# Autodesk Inventor assembly: 6 Plaction with bearings, pulleys and spacers
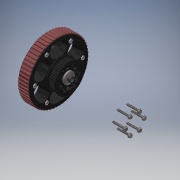
[picture p0: Inventor's stored thumbnail of the model, 180x180]
Saved by Autodesk Inventor 2018 (Build 220112000, 112)
## iProperties
Created: 2020-01-18
Part Number: 6 Plaction with bearings, pulleys and spacers
Document SubType Name: Assembly
Designer: maste
Author: maste
Revision Number: ANY
## Documents named in this file (7)
- \\studenthome\students\S-2512711\GitHub\2020CAD\Drivebase AM14U1\Part Files\6 Plaction with bearings, pulleys and spacers.iam
- \\studenthome\students\S-2512711\GitHub\2020CAD\Drivebase AM14U1\Part Files\42 tooth HTD Pulley half 2014.ipt
- \\studenthome\students\S-2512711\GitHub\2020CAD\Drivebase AM14U1\Part Files\1614Z Bearing.ipt
- \\studenthome\students\S-2512711\GitHub\2020CAD\Drivebase AM14U1\Part Files\10-24 Hex Washer Rolling x 1.25_93882A213.ipt
- \\studenthome\students\S-2512711\GitHub\2020CAD\Drivebase AM14U1\Part Files\am-1306 spacer 0280 WashersUSA 13RS052001.ipt
- \\studenthome\students\S-2512711\GitHub\2020CAD\Gabriel Inventor Files (Shooter, Drivebase)\Drivebase Assembly\Part Files\am-3316 6 inch Plaction Wheel with Roughtop.iam
- \\studenthome\students\S-2512711\GitHub\2020CAD\Gabriel Inventor Files (Shooter, Drivebase)\Drivebase Assembly\Part Files\Plaction wheel spacer.ipt
## Components (13 placed, 13 different names)
1. 42 tooth HTD Pulley half 2014_68 — Mate:3, Mate:4, Mate:5, Mate:14
2. 42 tooth HTD Pulley half 2014_69 — Mate:3, Mate:4, Mate:5, Mate:6, Mate:7, Mate:12, Mate:13
3. 1614Z Bearing_70 — Mate:6, Mate:7, Mate:8, Mate:9
4. 10-24 Hex Washer Rolling x 1.25_93882A213_71
5. 10-24 Hex Washer Rolling x 1.25_93882A213_72
6. 10-24 Hex Washer Rolling x 1.25_93882A213_73
7. 10-24 Hex Washer Rolling x 1.25_93882A213_74
8. 10-24 Hex Washer Rolling x 1.25_93882A213_75
9. 10-24 Hex Washer Rolling x 1.25_93882A213_76
10. am-1306 spacer 0280 WashersUSA 13RS052001_77 — Mate:8, Mate:9
11. 1614Z Bearing_78 — Mate:1, Mate:2, Mate:10, Mate:11
12. am-1307 850 long 380 id_79 — Mate:10, Mate:11
13. am-3316 6 inch Plaction Wheel with Roughtop:1 [sub-assembly] — Mate:1, Mate:2, Mate:12, Mate:13, Mate:14
## Relationships (14: Mate 14)
- Mate:1: 1614Z Bearing_78 ↔ am-3316 6 inch Plaction Wheel with Roughtop:1
- Mate:2: 1614Z Bearing_78 ↔ am-3316 6 inch Plaction Wheel with Roughtop:1
- Mate:3: 42 tooth HTD Pulley half 2014_68 ↔ 42 tooth HTD Pulley half 2014_69
- Mate:4: 42 tooth HTD Pulley half 2014_68 ↔ 42 tooth HTD Pulley half 2014_69
- Mate:5: 42 tooth HTD Pulley half 2014_68 ↔ 42 tooth HTD Pulley half 2014_69
- Mate:6: 42 tooth HTD Pulley half 2014_69 ↔ 1614Z Bearing_70
- Mate:7: 42 tooth HTD Pulley half 2014_69 ↔ 1614Z Bearing_70
- Mate:8: 1614Z Bearing_70 ↔ am-1306 spacer 0280 WashersUSA 13RS052001_77
- Mate:9: 1614Z Bearing_70 ↔ am-1306 spacer 0280 WashersUSA 13RS052001_77
- Mate:10: 1614Z Bearing_78 ↔ am-1307 850 long 380 id_79
- Mate:11: 1614Z Bearing_78 ↔ am-1307 850 long 380 id_79
- Mate:12: 42 tooth HTD Pulley half 2014_69 ↔ am-3316 6 inch Plaction Wheel with Roughtop:1
- Mate:13: 42 tooth HTD Pulley half 2014_69 ↔ am-3316 6 inch Plaction Wheel with Roughtop:1
- Mate:14: 42 tooth HTD Pulley half 2014_68 ↔ am-3316 6 inch Plaction Wheel with Roughtop:1
